# Autodesk Inventor assembly: Driveopen2
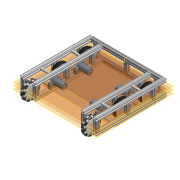
[picture p0: Inventor's stored thumbnail of the model, 180x180]
Saved by Autodesk Inventor 2013 (Build 170138000, 138)
## iProperties
Created: 2013-09-22
Part Number: Driveopen2
Document SubType Name: Assembly
Designer: Family Room
Mass: 858.54 g
Surface Area: 8628.43 cm^2
Volume: 788.69 cm^3
Density: 1.08856 g/cm^3
Author: Family Room
## Documents named in this file (9)
- C:\Users\rihoobler\Documents\GitHub\2013-2014_BlockParty\CAD\Drive\Final Drive Complete\Driveopen2.iam
- C:\Users\rihoobler\Documents\GitHub\2013-2014_BlockParty\CAD\Drive\Final Drive Complete\Frame Layer open.iam
- C:\Users\rihoobler\Documents\GitHub\2013-2014_BlockParty\CAD\Drive\Final Drive Complete\Verticle support.ipt
- C:\Users\rihoobler\Documents\GitHub\2013-2014_BlockParty\CAD\Drive\Final Drive Complete\axel support.ipt
- C:\Users\rihoobler\Documents\GitHub\2013-2014_BlockParty\CAD\Drive\Final Drive Complete\Tetrix Wheel 4 in omni.ipt
- C:\Users\rihoobler\Documents\GitHub\2013-2014_BlockParty\CAD\Drive\Final Drive Complete\Tetrix wheel 4 in.ipt
- C:\Users\rihoobler\Documents\GitHub\2013-2014_BlockParty\CAD\Drive\Final Drive Complete\pvc holder.ipt
- C:\Users\rihoobler\Documents\GitHub\2013-2014_BlockParty\CAD\Drive\Final Drive Complete\Motor Mount.ipt
- C:\Users\rihoobler\Documents\GitHub\2013-2014_BlockParty\CAD\Drive\Final Drive Complete\Motor.iam
## Components (41 placed, 8 different names)
1. Frame Layer open:1 [sub-assembly] — Mate:3, Flush:5, Mate:4, Flush:6, Flush:9, Mate:6, Flush:11, Mate:12, Flush:12, Flush:13, Mate:13, Flush:14, Flush:15, Mate:14, Flush:16, Flush:17, Mate:15, Angle:1, Flush:18, Mate:17, Angle:2, Mate:18, Mate:19, Flush:19, Mate:20, Flush:21, Mate:21, Flush:23, Flush:24, Mate:22, Flush:25, Mate:23, Flush:27, Mate:24, Flush:29, Mate:25, Flush:31, Mate:32, Mate:35, Mate:37, Mate:38, Mate:72, Flush:50, Mate:74, Flush:51, Mate:76, Flush:52, Flush:53, Mate:77, Flush:60, Mate:98, Mate:99, Mate:101, Mate:102, Mate:103, Mate:104, Mate:105
2. Frame Layer open:2 [sub-assembly] — Flush:9, Flush:10, Mate:33, Mate:34, Mate:36, Mate:82, Mate:85, Mate:86, Mate:87, Mate:88, Mate:89, Mate:90, Mate:91, Mate:92, Mate:93, Mate:94, Mate:95, Mate:96, Mate:97
3. Verticle support:3 — Mate:4, Flush:6, Flush:10, Mate:7, Mate:97
4. Verticle support:4 — Mate:3, Flush:5
5. Verticle support:5 — Mate:6, Flush:11, Mate:7
6. axel support:1 — Mate:14, Flush:16, Flush:17, Mate:27
7. axel support:2 — Mate:25, Flush:31, Flush:32, Mate:31
8. axel support:3 — Mate:21, Flush:23, Flush:24, Mate:82, Mate:83
9. axel support:4 — Mate:12, Flush:12, Flush:13, Mate:16, Mate:26, Mate:84
10. axel support:5 — Mate:13, Flush:14, Flush:15
11. axel support:6 — Mate:15, Angle:1, Flush:18, Mate:16, Flush:20, Flush:26, Mate:28, Mate:73
12. axel support:7 — Mate:17, Angle:2, Mate:18, Flush:22, Flush:28, Mate:29, Mate:75
13. axel support:8 — Mate:19, Flush:19, Flush:20
14. axel support:9 — Mate:20, Flush:21, Flush:22
15. axel support:10 — Mate:24, Flush:29, Flush:30, Mate:30
16. axel support:11 — Mate:22, Flush:25, Flush:26, Flush:30
17. axel support:12 — Mate:23, Flush:27, Flush:28, Flush:32
18. Tetrix Wheel 4 in omni:1 — Mate:26, Mate:40, Mate:42, Mate:43, Flush:36, Mate:84
19. Tetrix Wheel 4 in omni:2 — Mate:27, Mate:41, Mate:44, Mate:45, Mate:83
20. Tetrix wheel 4 in:1 — Mate:31, Flush:34
21. Tetrix wheel 4 in:2 — Mate:30, Flush:34, Flush:35, Mate:109
22. Tetrix wheel 4 in:3 — Mate:28, Flush:36, Flush:37, Mate:107
23. Tetrix wheel 4 in:4 — Mate:29, Flush:37, Mate:108
24. pvc holder:1 — Mate:36, Mate:90, Mate:94
25. pvc holder:2 — Mate:89, Mate:91, Mate:92, Mate:93, Flush:63
26. pvc holder:3 — Mate:38, Flush:63, Mate:103, Mate:104, Mate:105
27. pvc holder:4 — Mate:37, Mate:98, Mate:99, Mate:106
28. pvc holder:5 — Mate:33, Mate:85, Mate:86, Mate:88, Mate:95
29. pvc holder:6 — Mate:32, Mate:101, Mate:106
30. pvc holder:7 — Mate:34, Mate:87, Mate:96
31. pvc holder:8 — Mate:35, Mate:102
32. Tetrix Wheel 4 in omni:3 — Mate:40, Mate:42, Mate:43
33. Tetrix Wheel 4 in omni:4 — Mate:41, Mate:44, Mate:45, Flush:35
34. Motor Mount:1 — Mate:72, Flush:50, Mate:73, Flush:55, Mate:78, Flush:57
35. Motor Mount:2 — Mate:74, Flush:51, Mate:75, Flush:54, Mate:79, Flush:56
36. Motor Mount:3 — Mate:76, Flush:52, Flush:55, Mate:80, Flush:58
37. Motor Mount:4 — Flush:53, Mate:77, Flush:54, Mate:81, Flush:59
38. Motor:1 [sub-assembly] — Mate:78, Flush:57
39. Motor:2 [sub-assembly] — Mate:79, Flush:56
40. Motor:3 [sub-assembly] — Mate:80, Flush:58
41. Motor:4 [sub-assembly] — Mate:81, Flush:59
## Relationships (121: Mate 74, Flush 45, Angle 2)
- Mate:3: Frame Layer open:1 ↔ Verticle support:4
- Flush:5: Frame Layer open:1 ↔ Verticle support:4
- Mate:4: Frame Layer open:1 ↔ Verticle support:3
- Flush:6: Frame Layer open:1 ↔ Verticle support:3
- Flush:9: Frame Layer open:1 ↔ Frame Layer open:2
- Flush:10: Frame Layer open:2 ↔ Verticle support:3
- Mate:6: Frame Layer open:1 ↔ Verticle support:5
- Flush:11: Frame Layer open:1 ↔ Verticle support:5
- Mate:7 (156.8526 mm): Verticle support:3 ↔ Verticle support:5
- Mate:12: Frame Layer open:1 ↔ axel support:4
- Flush:12: Frame Layer open:1 ↔ axel support:4
- Flush:13: Frame Layer open:1 ↔ axel support:4
- Mate:13: Frame Layer open:1 ↔ axel support:5
- Flush:14: Frame Layer open:1 ↔ axel support:5
- Flush:15: Frame Layer open:1 ↔ axel support:5
- Mate:14: Frame Layer open:1 ↔ axel support:1
- Flush:16: Frame Layer open:1 ↔ axel support:1
- Flush:17: Frame Layer open:1 ↔ axel support:1
- Mate:15: Frame Layer open:1 ↔ axel support:6
- Angle:1 (0 deg): Frame Layer open:1 ↔ axel support:6
- Flush:18: Frame Layer open:1 ↔ axel support:6
- Mate:16 (158.75 mm): axel support:4 ↔ axel support:6
- Mate:17: Frame Layer open:1 ↔ axel support:7
- Angle:2 (0 deg): Frame Layer open:1 ↔ axel support:7
- Mate:18: Frame Layer open:1 ↔ axel support:7
- Mate:19: Frame Layer open:1 ↔ axel support:8
- Flush:19: Frame Layer open:1 ↔ axel support:8
- Flush:20: axel support:6 ↔ axel support:8
- Mate:20: Frame Layer open:1 ↔ axel support:9
- Flush:21: Frame Layer open:1 ↔ axel support:9
- Flush:22: axel support:7 ↔ axel support:9
- Mate:21: Frame Layer open:1 ↔ axel support:3
- Flush:23: Frame Layer open:1 ↔ axel support:3
- Flush:24: Frame Layer open:1 ↔ axel support:3
- Mate:22: Frame Layer open:1 ↔ axel support:11
- Flush:25: Frame Layer open:1 ↔ axel support:11
- Flush:26: axel support:6 ↔ axel support:11
- Mate:23: Frame Layer open:1 ↔ axel support:12
- Flush:27: Frame Layer open:1 ↔ axel support:12
- Flush:28: axel support:7 ↔ axel support:12
- Mate:24: Frame Layer open:1 ↔ axel support:10
- Flush:29: Frame Layer open:1 ↔ axel support:10
- Flush:30: axel support:10 ↔ axel support:11
- Mate:25: Frame Layer open:1 ↔ axel support:2
- Flush:31: Frame Layer open:1 ↔ axel support:2
- Flush:32: axel support:2 ↔ axel support:12
- Mate:26: axel support:4 ↔ Tetrix Wheel 4 in omni:1
- Mate:27: axel support:1 ↔ Tetrix Wheel 4 in omni:2
- Mate:28: axel support:6 ↔ Tetrix wheel 4 in:3
- Mate:29: axel support:7 ↔ Tetrix wheel 4 in:4
- Mate:30: axel support:10 ↔ Tetrix wheel 4 in:2
- Mate:31: axel support:2 ↔ Tetrix wheel 4 in:1
- Mate:32: Frame Layer open:1 ↔ pvc holder:6
- Mate:33: Frame Layer open:2 ↔ pvc holder:5
- Mate:34: Frame Layer open:2 ↔ pvc holder:7
- Mate:35: Frame Layer open:1 ↔ pvc holder:8
- Mate:36: Frame Layer open:2 ↔ pvc holder:1
- Mate:37: Frame Layer open:1 ↔ pvc holder:4
- Mate:38: Frame Layer open:1 ↔ pvc holder:3
- Mate:40: Tetrix Wheel 4 in omni:1 ↔ Tetrix Wheel 4 in omni:3
- Mate:41: Tetrix Wheel 4 in omni:2 ↔ Tetrix Wheel 4 in omni:4
- Mate:42: Tetrix Wheel 4 in omni:1 ↔ Tetrix Wheel 4 in omni:3
- Mate:43: Tetrix Wheel 4 in omni:1 ↔ Tetrix Wheel 4 in omni:3
- Mate:44: Tetrix Wheel 4 in omni:2 ↔ Tetrix Wheel 4 in omni:4
- Mate:45: Tetrix Wheel 4 in omni:2 ↔ Tetrix Wheel 4 in omni:4
- Flush:34: Tetrix wheel 4 in:1 ↔ Tetrix wheel 4 in:2
- Flush:35: Tetrix wheel 4 in:2 ↔ Tetrix Wheel 4 in omni:4
- Flush:36: Tetrix Wheel 4 in omni:1 ↔ Tetrix wheel 4 in:3
- Flush:37: Tetrix wheel 4 in:3 ↔ Tetrix wheel 4 in:4
- Mate:72: Frame Layer open:1 ↔ Motor Mount:1
- Flush:50: Frame Layer open:1 ↔ Motor Mount:1
- Mate:73 (25.4 mm): axel support:6 ↔ Motor Mount:1
- Mate:74: Frame Layer open:1 ↔ Motor Mount:2
- Flush:51: Frame Layer open:1 ↔ Motor Mount:2
- Mate:75 (25.4 mm): axel support:7 ↔ Motor Mount:2
- Mate:76: Frame Layer open:1 ↔ Motor Mount:3
- Flush:52: Frame Layer open:1 ↔ Motor Mount:3
- Flush:53: Frame Layer open:1 ↔ Motor Mount:4
- Mate:77: Frame Layer open:1 ↔ Motor Mount:4
- Flush:54: Motor Mount:2 ↔ Motor Mount:4
- Flush:55: Motor Mount:1 ↔ Motor Mount:3
- Mate:78: Motor Mount:1 ↔ Motor:1
- Mate:79: Motor Mount:2 ↔ Motor:2
- Mate:80: Motor Mount:3 ↔ Motor:3
- Mate:81: Motor Mount:4 ↔ Motor:4
- Flush:56: Motor Mount:2 ↔ Motor:2
- Flush:57: Motor Mount:1 ↔ Motor:1
- Flush:58: Motor Mount:3 ↔ Motor:3
- Flush:59: Motor Mount:4 ↔ Motor:4
- Flush:60 (12.7 mm): Frame Layer open:1
- Flush:61 (17.907 mm)
- Flush:62 (-17.907 mm)
- Mate:82: Frame Layer open:2 ↔ axel support:3
- Mate:83 (12.7 mm): axel support:3 ↔ Tetrix Wheel 4 in omni:2
- Mate:84 (12.7 mm): axel support:4 ↔ Tetrix Wheel 4 in omni:1
- Mate:85: Frame Layer open:2 ↔ pvc holder:5
- Mate:86: Frame Layer open:2 ↔ pvc holder:5
- Mate:87 (-130.175 mm): Frame Layer open:2 ↔ pvc holder:7
- Mate:88 (-307.975 mm): Frame Layer open:2 ↔ pvc holder:5
- Mate:89 (-130.175 mm): Frame Layer open:2 ↔ pvc holder:2
- Mate:90 (-307.975 mm): Frame Layer open:2 ↔ pvc holder:1
- Mate:91: Frame Layer open:2 ↔ pvc holder:2
- Mate:92: Frame Layer open:2 ↔ pvc holder:2
- Mate:93 (-8.128 mm): Frame Layer open:2 ↔ pvc holder:2
- Mate:94 (-8.128 mm): Frame Layer open:2 ↔ pvc holder:1
- Mate:95 (-8.128 mm): Frame Layer open:2 ↔ pvc holder:5
- Mate:96 (-8.128 mm): Frame Layer open:2 ↔ pvc holder:7
- Mate:97: Frame Layer open:2 ↔ Verticle support:3
- Mate:98: Frame Layer open:1 ↔ pvc holder:4
- Mate:99 (-3.302 mm): Frame Layer open:1 ↔ pvc holder:4
- Mate:101 (-3.302 mm): Frame Layer open:1 ↔ pvc holder:6
- Mate:102 (8.128 mm): Frame Layer open:1 ↔ pvc holder:8
- Flush:63: pvc holder:2 ↔ pvc holder:3
- Mate:103: Frame Layer open:1 ↔ pvc holder:3
- Mate:104 (-120.65 mm): Frame Layer open:1 ↔ pvc holder:3
- Mate:105: Frame Layer open:1 ↔ pvc holder:3
- Mate:106: pvc holder:4 ↔ pvc holder:6
- Mate:107: Tetrix wheel 4 in:3
- Mate:108: Tetrix wheel 4 in:4
- Mate:109: Tetrix wheel 4 in:2
- Flush:64 (48.7934 mm)
